# Autodesk Inventor assembly: LargeSkirtWall
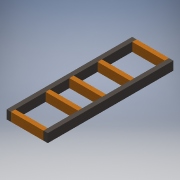
[picture p0: Inventor's stored thumbnail of the model, 180x180]
Saved by Autodesk Inventor 2016 (Build 200138000, 138)
## iProperties
Created: 2016-06-15
Part Number: LargeSkirtWall
Document SubType Name: Assembly
Designer: cutrones
Author: cutrones
## Documents named in this file (3)
- C:\Users\cutrones\Desktop\MotionBase\CAD\MotionBaseCAD\BaseSkirt\LargeSkirtWall.iam
- C:\Users\cutrones\Desktop\MotionBase\CAD\MotionBaseCAD\BaseSkirt\LargeHorizBeam.ipt
- C:\Users\cutrones\Desktop\MotionBase\CAD\MotionBaseCAD\BaseSkirt\VertBeam.ipt
## Components (7 placed, 2 different names)
1. LargeHorizBeam:5 — Flush:3, Mate:2, Flush:4
2. LargeHorizBeam:6 — Flush:1, Mate:1, Flush:2, Flush:5, Mate:3, Flush:6, Mate:4, Mate:5, Flush:7, Flush:8, Mate:8, Flush:9
3. VertBeam:9 — Flush:5, Mate:3, Flush:6, Mate:7
4. VertBeam:10 — Mate:5, Flush:8, Mate:7
5. VertBeam:11 — Mate:4, Flush:7, Mate:6
6. VertBeam:12 — Flush:1, Mate:1, Flush:2, Flush:3, Mate:2, Flush:4, Mate:6, Mate:9
7. VertBeam:14 — Mate:8, Flush:9, Mate:9
## Relationships (18: Flush 9, Mate 9)
- Flush:1: LargeHorizBeam:6 ↔ VertBeam:12
- Mate:1: LargeHorizBeam:6 ↔ VertBeam:12
- Flush:2: LargeHorizBeam:6 ↔ VertBeam:12
- Flush:3: LargeHorizBeam:5 ↔ VertBeam:12
- Mate:2: LargeHorizBeam:5 ↔ VertBeam:12
- Flush:4: LargeHorizBeam:5 ↔ VertBeam:12
- Flush:5: LargeHorizBeam:6 ↔ VertBeam:9
- Mate:3: LargeHorizBeam:6 ↔ VertBeam:9
- Flush:6: LargeHorizBeam:6 ↔ VertBeam:9
- Mate:4: LargeHorizBeam:6 ↔ VertBeam:11
- Mate:5: LargeHorizBeam:6 ↔ VertBeam:10
- Flush:7: LargeHorizBeam:6 ↔ VertBeam:11
- Flush:8: LargeHorizBeam:6 ↔ VertBeam:10
- Mate:6 (635 mm): VertBeam:11 ↔ VertBeam:12
- Mate:7 (355.6 mm): VertBeam:9 ↔ VertBeam:10
- Mate:8: LargeHorizBeam:6 ↔ VertBeam:14
- Flush:9: LargeHorizBeam:6 ↔ VertBeam:14
- Mate:9 (355.6 mm): VertBeam:12 ↔ VertBeam:14
